# Autodesk Inventor assembly: ensamble_general
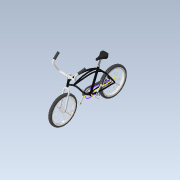
[picture p0: Inventor's stored thumbnail of the model, 180x180]
Saved by Autodesk Inventor 2021 (Build 250183000, 183)
## iProperties
Created: 2021-04-10
Part Number: ensamble_general
Document SubType Name: Assembly
Designer: j2seb
Author: j2seb
## Documents named in this file (10)
- G:\Unidades compartidas\APM\02 Inventor-Drive\ensamble_general.iam
- G:\Unidades compartidas\APM\02 Inventor-Drive\Marco_Bicicleta.iam
- G:\Unidades compartidas\APM\02 Inventor-Drive\Manubrio\Manubrio.ipt
- G:\Unidades compartidas\APM\02 Inventor-Drive\Ensamble_Llanta.iam
- G:\Unidades compartidas\APM\02 Inventor-Drive\sillin.iam
- G:\Unidades compartidas\APM\02 Inventor-Drive\caja_pedalera.iam
- G:\Unidades compartidas\APM\02 Inventor-Drive\Transmision\Cadena.iam
- G:\Unidades compartidas\APM\02 Inventor-Drive\Transmision\Design Accelerator\Roller Chain Sprocket11.ipt
- G:\Unidades compartidas\APM\02 Inventor-Drive\cubrecadena.ipt
- G:\Unidades compartidas\APM\02 Inventor-Drive\llanta trasera.iam
## Components (9 placed, 9 different names)
1. Marco_Bicicleta:1 [sub-assembly] — Coincidencia:3, Flush:1, Cylindrical:2, Mate:5, Coincidencia:6, Coincidencia:7, Mate:8, Mate:9
2. Manubrio:1 — Flush:1, Cylindrical:3
3. Ensamble_Llanta:2 [sub-assembly] — Cylindrical:3
4. sillin:1 [sub-assembly] — Cylindrical:2, Mate:5
5. caja_pedalera:1 [sub-assembly] — Coincidencia:6, Coincidencia:7
6. Cadena:1 [sub-assembly] — Mate:11, Mate:12
7. Roller Chain Sprocket1:1 — Mate:11, Mate:13
8. cubrecadena:1 — Mate:15
9. llanta trasera:1 [sub-assembly]
## Relationships (15: Mate 11, CylindricalJoint 2, Angle 1, Flush 1)
- [Mate]: Marco_Bicicleta:1 ↔ llanta trasera:1
- Coincidencia:3 [Mate]: Marco_Bicicleta:1
- Ángulo:1 [Angle] (0 deg)
- Flush:1 (-55.052 mm): Marco_Bicicleta:1 ↔ Manubrio:1
- Cylindrical:2: Marco_Bicicleta:1 ↔ sillin:1
- Mate:5 (-50 mm): Marco_Bicicleta:1 ↔ sillin:1
- Cylindrical:3: Manubrio:1 ↔ Ensamble_Llanta:2
- Coincidencia:6 [Mate]: Marco_Bicicleta:1 ↔ caja_pedalera:1
- Coincidencia:7 [Mate]: Marco_Bicicleta:1 ↔ caja_pedalera:1
- Mate:8: Marco_Bicicleta:1
- Mate:9: Marco_Bicicleta:1
- Mate:11: Cadena:1 ↔ Roller Chain Sprocket1:1
- Mate:12: Cadena:1
- Mate:13: Roller Chain Sprocket1:1
- Mate:15: cubrecadena:1
## Named parameters: DExtTub = 42.164 mm, DintTub = 35.052 mm, DIntTubTen = 28 mm, DAguUniMarcoLlanta = 4 mm
